# Autodesk Inventor assembly: Head
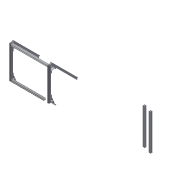
[picture p0: Inventor's stored thumbnail of the model, 180x180]
Saved by Autodesk Inventor 2014 SP1 (Build 180222100, 222)
## iProperties
Created: 2015-02-11
Part Number: Head
Document SubType Name: Assembly
Designer: Simen
Author: Simen
## Documents named in this file (8)
- C:\Users\Simen\Documents\git\Eit\skjellet\Head.iam
- C:\Users\Simen\Documents\git\Eit\skjellet\KHFS5_2020_350.ipt
- C:\Users\Simen\Documents\git\Eit\skjellet\HBL45TS6hbl45ts6.ipt
- C:\Users\Simen\Documents\git\Eit\skjellet\HBL135TS6.iam
- C:\Users\Simen\Documents\git\Eit\skjellet\KHFS5_2020_386.ipt
- C:\Users\Simen\Documents\git\Eit\skjellet\KHFS5_2020_391.ipt
- C:\Users\Simen\Documents\git\Eit\skjellet\KHFS5_2020_287,5.ipt
- C:\Users\Simen\Documents\git\Eit\skjellet\KHFS5_2020_143,5.ipt
## Components (16 placed, 3 different names)
1. HBL45TS6hbl45ts6:1 — Mate:1, Flush:1, Mate:2, Mate:42, Flush:38, Mate:43
2. KHFS5-2020-4000:1 — Mate:1, Flush:1, Mate:2, Mate:6, Flush:5, Mate:7, Mate:40, Flush:36, Flush:37
3. HBL135TS6:1 [sub-assembly] — Mate:6, Flush:5, Mate:7, Mate:47, Flush:44
4. KHFS5-2020-4000:7 — Mate:39, Flush:34, Flush:35, Mate:53, Flush:50, Flush:51
5. HBL45TS6hbl45ts6:2 — Mate:41, Flush:39, Mate:44
6. HBL135TS6:2 [sub-assembly] — Mate:49, Flush:45
7. KHFS5-2020-4000:17 — Mate:39, Flush:34, Flush:35, Mate:40, Flush:36, Flush:37
8. KHFS5-2020-4000:18 — Mate:41, Flush:39, Mate:44, Flush:41, Mate:46, Flush:43
9. KHFS5-2020-4000:19 — Mate:42, Flush:38, Mate:43, Mate:45, Flush:40, Flush:42
10. KHFS5-2020-4000:21 — Flush:41, Mate:46, Flush:43, Mate:50, Mate:51, Mate:52
11. KHFS5-2020-4000:22 — Mate:45, Flush:40, Flush:42, Mate:48, Flush:46, Flush:47, Flush:48, Flush:49
12. KHFS5-2020-4000:24 — Mate:47, Flush:44, Mate:48
13. KHFS5-2020-4000:25 — Mate:49, Flush:45, Mate:50
14. KHFS5-2020-4000:26 — Mate:51, Flush:47, Flush:48
15. KHFS5-2020-4000:27 — Mate:52, Flush:46, Flush:49
16. KHFS5-2020-4000:28 — Mate:53, Flush:50, Flush:51
## Relationships (45: Mate 23, Flush 22)
- Mate:1: HBL45TS6hbl45ts6:1 ↔ KHFS5-2020-4000:1
- Flush:1: HBL45TS6hbl45ts6:1 ↔ KHFS5-2020-4000:1
- Mate:2: HBL45TS6hbl45ts6:1 ↔ KHFS5-2020-4000:1
- Mate:6: KHFS5-2020-4000:1 ↔ HBL135TS6:1
- Flush:5: KHFS5-2020-4000:1 ↔ HBL135TS6:1
- Mate:7: KHFS5-2020-4000:1 ↔ HBL135TS6:1
- [Mate]: KHFS5-2020-4000:7 ↔ HBL45TS6hbl45ts6:2
- [Flush]: KHFS5-2020-4000:7 ↔ HBL45TS6hbl45ts6:2
- [Mate]: KHFS5-2020-4000:7 ↔ HBL45TS6hbl45ts6:2
- [Mate]: KHFS5-2020-4000:7 ↔ HBL135TS6:2
- [Flush]: KHFS5-2020-4000:7 ↔ HBL135TS6:2
- [Mate]: KHFS5-2020-4000:7 ↔ HBL135TS6:2
- Mate:39: KHFS5-2020-4000:7 ↔ KHFS5-2020-4000:17
- Flush:34: KHFS5-2020-4000:7 ↔ KHFS5-2020-4000:17
- Flush:35: KHFS5-2020-4000:7 ↔ KHFS5-2020-4000:17
- Mate:40: KHFS5-2020-4000:1 ↔ KHFS5-2020-4000:17
- Flush:36: KHFS5-2020-4000:1 ↔ KHFS5-2020-4000:17
- Flush:37: KHFS5-2020-4000:1 ↔ KHFS5-2020-4000:17
- Mate:41: HBL45TS6hbl45ts6:2 ↔ KHFS5-2020-4000:18
- Mate:42: HBL45TS6hbl45ts6:1 ↔ KHFS5-2020-4000:19
- Flush:38: HBL45TS6hbl45ts6:1 ↔ KHFS5-2020-4000:19
- Flush:39: HBL45TS6hbl45ts6:2 ↔ KHFS5-2020-4000:18
- Mate:43: HBL45TS6hbl45ts6:1 ↔ KHFS5-2020-4000:19
- Mate:44: HBL45TS6hbl45ts6:2 ↔ KHFS5-2020-4000:18
- Mate:45: KHFS5-2020-4000:19 ↔ KHFS5-2020-4000:22
- Flush:40: KHFS5-2020-4000:19 ↔ KHFS5-2020-4000:22
- Flush:41: KHFS5-2020-4000:18 ↔ KHFS5-2020-4000:21
- Mate:46: KHFS5-2020-4000:18 ↔ KHFS5-2020-4000:21
- Flush:42: KHFS5-2020-4000:19 ↔ KHFS5-2020-4000:22
- Flush:43: KHFS5-2020-4000:18 ↔ KHFS5-2020-4000:21
- Mate:47: HBL135TS6:1 ↔ KHFS5-2020-4000:24
- Flush:44: HBL135TS6:1 ↔ KHFS5-2020-4000:24
- Mate:48: KHFS5-2020-4000:22 ↔ KHFS5-2020-4000:24
- Mate:49: HBL135TS6:2 ↔ KHFS5-2020-4000:25
- Flush:45: HBL135TS6:2 ↔ KHFS5-2020-4000:25
- Mate:50: KHFS5-2020-4000:21 ↔ KHFS5-2020-4000:25
- Mate:51: KHFS5-2020-4000:21 ↔ KHFS5-2020-4000:26
- Mate:52: KHFS5-2020-4000:21 ↔ KHFS5-2020-4000:27
- Flush:46: KHFS5-2020-4000:22 ↔ KHFS5-2020-4000:27
- Flush:47: KHFS5-2020-4000:22 ↔ KHFS5-2020-4000:26
- Flush:48: KHFS5-2020-4000:22 ↔ KHFS5-2020-4000:26
- Flush:49: KHFS5-2020-4000:22 ↔ KHFS5-2020-4000:27
- Mate:53: KHFS5-2020-4000:7 ↔ KHFS5-2020-4000:28
- Flush:50: KHFS5-2020-4000:7 ↔ KHFS5-2020-4000:28
- Flush:51: KHFS5-2020-4000:7 ↔ KHFS5-2020-4000:28
## Named parameters: d13_d0 = 0 mm, d14_d1 = 0 mm, d15_d2 = 0 mm, d16_d10 = 0 mm, d17_d11 = 0 mm, d18_d12 = 0 mm
